# Autodesk Inventor assembly: Mounting
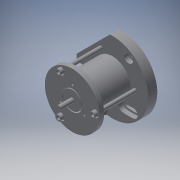
[picture p0: Inventor's stored thumbnail of the model, 180x180]
Saved by Autodesk Inventor 2018 (Build 220112000, 112)
## iProperties
Created: 2018-03-20
Part Number: Mounting
Document SubType Name: Assembly
Designer: P301319
Author: P301319
## Documents named in this file (5)
- E:\2018 CNC Lathe\Encoder Packed\Mounting.iam
- E:\2018 CNC Lathe\Encoder Packed\Working Encoder.iam
- E:\2018 CNC Lathe\Encoder Packed\Encoder Mount Front.ipt
- E:\2018 CNC Lathe\Encoder Packed\Encoder Mount Base.ipt
- E:\2018 CNC Lathe\Encoder Packed\Fake Bolt.ipt
## Components (6 placed, 4 different names)
1. Working Encoder:1 [sub-assembly] — Mate:1, Mate:2, Mate:7, Mate:9, Mate:16, Mate:17
2. Encoder Mount Base:1 — Mate:1, Mate:2, Mate:4, Mate:6, Mate:8, Angle:1
3. Encoder Mount Front:1 — Mate:7, Mate:8, Mate:9, Mate:10, Mate:11, Mate:12, Mate:13, Mate:14, Mate:15, Mate:16
4. Fake Bolt:1 — Mate:10, Mate:15
5. Fake Bolt:2 — Mate:11, Mate:14
6. Fake Bolt:3 — Mate:12, Mate:13
## Relationships (16: Mate 15, Angle 1)
- Mate:1: Working Encoder:1 ↔ Encoder Mount Base:1
- Mate:2: Working Encoder:1 ↔ Encoder Mount Base:1
- Mate:4: Encoder Mount Base:1
- Mate:6: Encoder Mount Base:1
- Mate:7: Working Encoder:1 ↔ Encoder Mount Front:1
- Mate:8: Encoder Mount Base:1 ↔ Encoder Mount Front:1
- Mate:9: Working Encoder:1 ↔ Encoder Mount Front:1
- Mate:10: Encoder Mount Front:1 ↔ Fake Bolt:1
- Mate:11: Encoder Mount Front:1 ↔ Fake Bolt:2
- Mate:12: Encoder Mount Front:1 ↔ Fake Bolt:3
- Mate:13: Encoder Mount Front:1 ↔ Fake Bolt:3
- Mate:14: Encoder Mount Front:1 ↔ Fake Bolt:2
- Mate:15: Encoder Mount Front:1 ↔ Fake Bolt:1
- Mate:16: Working Encoder:1 ↔ Encoder Mount Front:1
- Angle:1 (135 deg): Encoder Mount Base:1
- Mate:17: Working Encoder:1
